# Autodesk Inventor assembly: box1
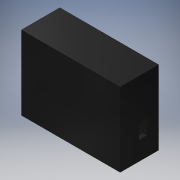
[picture p0: Inventor's stored thumbnail of the model, 180x180]
Saved by Autodesk Inventor 2019 (Build 230136000, 136)
## iProperties
Created: 2018-06-07
Part Number: box1
Document SubType Name: Assembly
Designer: stra92745
Author: stra92745
## Documents named in this file (7)
- C:\Users\stra92745\source\Workspaces\et-sys-dev\ET Internal Projects\SSTrolley\Dev\hardware\boxes\box1\box1.iam
- C:\Users\stra92745\source\Workspaces\et-sys-dev\ET Internal Projects\SSTrolley\Dev\hardware\boxes\box1\back.ipt
- C:\Users\stra92745\source\Workspaces\et-sys-dev\ET Internal Projects\SSTrolley\Dev\hardware\boxes\box1\bottom.ipt
- C:\Users\stra92745\source\Workspaces\et-sys-dev\ET Internal Projects\SSTrolley\Dev\hardware\boxes\box1\front.ipt
- C:\Users\stra92745\source\Workspaces\et-sys-dev\ET Internal Projects\SSTrolley\Dev\hardware\boxes\box1\left.ipt
- C:\Users\stra92745\source\Workspaces\et-sys-dev\ET Internal Projects\SSTrolley\Dev\hardware\boxes\box1\right.ipt
- C:\Users\stra92745\source\Workspaces\et-sys-dev\ET Internal Projects\SSTrolley\Dev\hardware\boxes\box1\top.ipt
## Components (6 placed, 6 different names)
1. back:1 — Mate:4, Mate:5, Mate:6, Mate:16, Mate:17
2. bottom:1 — Mate:1, Mate:2, Mate:3, Mate:4, Mate:5, Mate:6, Mate:7, Mate:8, Mate:9, Mate:10, Mate:11, Mate:12, Mate:13, Mate:14, Mate:15
3. front:1 — Mate:7, Mate:8, Mate:9
4. left:1 — Mate:10, Mate:11, Mate:12
5. right:1 — Mate:13, Mate:14, Mate:15, Mate:18
6. top:1 — Mate:16, Mate:17, Mate:18
## Relationships (18: Mate 18)
- Mate:1: bottom:1
- Mate:2: bottom:1
- Mate:3: bottom:1
- Mate:4: back:1 ↔ bottom:1
- Mate:5: back:1 ↔ bottom:1
- Mate:6: back:1 ↔ bottom:1
- Mate:7: bottom:1 ↔ front:1
- Mate:8: bottom:1 ↔ front:1
- Mate:9: bottom:1 ↔ front:1
- Mate:10: bottom:1 ↔ left:1
- Mate:11: bottom:1 ↔ left:1
- Mate:12: bottom:1 ↔ left:1
- Mate:13: bottom:1 ↔ right:1
- Mate:14: bottom:1 ↔ right:1
- Mate:15: bottom:1 ↔ right:1
- Mate:16: back:1 ↔ top:1
- Mate:17: back:1 ↔ top:1
- Mate:18: right:1 ↔ top:1
